# Autodesk Inventor assembly: ensamble_general
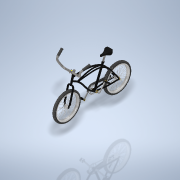
[picture p0: Inventor's stored thumbnail of the model, 180x180]
Saved by Autodesk Inventor 2021 (Build 250183000, 183)
## iProperties
Created: 2021-04-10
Part Number: ensamble_general
Document SubType Name: Assembly
Designer: j2seb
Author: j2seb
## Documents named in this file (17)
- C:\Users\leo7s\Documents\Universidad\03 APM\04 Gitrespository\Proyecto_APM\02 Inventor\ensamble_general.iam
- C:\Users\leo7s\Documents\Universidad\03 APM\04 Gitrespository\Proyecto_APM\02 Inventor\Marco_Bicicleta.iam
- C:\Users\leo7s\Documents\Universidad\03 APM\04 Gitrespository\Proyecto_APM\02 Inventor\Manubrio\Manubrio.ipt
- C:\Users\leo7s\Documents\Universidad\03 APM\04 Gitrespository\Proyecto_APM\02 Inventor\sillin.iam
- C:\Users\leo7s\Documents\Universidad\03 APM\04 Gitrespository\Proyecto_APM\02 Inventor\caja_pedalera.iam
- C:\Users\leo7s\Documents\Universidad\03 APM\04 Gitrespository\Proyecto_APM\02 Inventor\Transmision\Cadena.iam
- C:\Users\leo7s\Documents\Universidad\03 APM\04 Gitrespository\Proyecto_APM\02 Inventor\cubrecadena.ipt
- C:\Users\leo7s\Documents\Universidad\03 APM\04 Gitrespository\Proyecto_APM\02 Inventor\llanta trasera.iam
- C:\Users\leo7s\Documents\Universidad\03 APM\04 Gitrespository\Proyecto_APM\02 Inventor\llanta delantera.iam
- C:\Users\leo7s\Documents\Universidad\03 APM\04 Gitrespository\Proyecto_APM\02 Inventor\platina_1.ipt
- C:\Users\leo7s\Documents\Universidad\03 APM\04 Gitrespository\Proyecto_APM\02 Inventor\platina_2.ipt
- C:\Users\leo7s\Documents\Universidad\03 APM\04 Gitrespository\Proyecto_APM\02 Inventor\platina_3.ipt
- C:\Users\j2seb\OneDrive\Documents\Inventor\Content Center Files\R2021\es-ES\ISO 7045(1)\DIN EN ISO 7045 - M3 x 8 - 4.8 - H.ipt
- C:\Users\j2seb\OneDrive\Documents\Inventor\Content Center Files\R2021\es-ES\DIN 125-2  A\DIN 125-2 - A 3,2A.ipt
- C:\Users\j2seb\OneDrive\Documents\Inventor\Content Center Files\R2021\es-ES\DIN 439-2\DIN 439 - M3 x 0,5.ipt
- C:\Users\j2seb\OneDrive\Documents\Inventor\Content Center Files\R2021\es-ES\ISO 7045(2)\DIN EN ISO 7045 - M3 x 8 - 4.8 - Z.ipt
- C:\Users\leo7s\Documents\Universidad\03 APM\04 Gitrespository\Proyecto_APM\02 Inventor\platina_4.ipt
## Components (21 placed, 16 different names)
1. Marco_Bicicleta:1 [sub-assembly] — Flush:1, Cylindrical:2, Mate:5, Coincidencia:6, Coincidencia:7, Mate:8, Mate:9, Coincidencia:16, Coincidencia:19, Mate:20, Coincidencia:37
2. Manubrio:1 — Flush:1, Coincidencia:19, Mate:21
3. sillin:1 [sub-assembly] — Cylindrical:2, Mate:5
4. caja_pedalera:1 [sub-assembly] — Coincidencia:6, Coincidencia:7
5. Cadena:1 [sub-assembly] — Mate:12
6. cubrecadena:1 — Mate:15, Coincidencia:23, Nivelación:2, Coincidencia:24, Nivelación:3, Coincidencia:25, Coincidencia:29, Coincidencia:30, Coincidencia:31, Coincidencia:32, Nivelación:4
7. llanta trasera:1 [sub-assembly] — Coincidencia:16
8. llanta delantera:1 [sub-assembly] — Mate:20, Mate:22
9. platina_1:1 — Coincidencia:23, Nivelación:2, Coincidencia:26, Coincidencia:27, Coincidencia:28
10. platina_2:1 — Coincidencia:24, Nivelación:3, Nivelación:4, Coincidencia:34
11. platina_3:1 — Coincidencia:25, Coincidencia:33
12. DIN EN ISO 7045 H M3 x 8 - 4.8 - H:1 — Coincidencia:26, Coincidencia:27
13. DIN 125-2 A A 3,2:1 — Coincidencia:28, Coincidencia:29, Insertar:1
14. DIN 439-2 - reemplazado por DIN EN 24035/28675 M3:1 — Insertar:1
15. DIN EN ISO 7045 Z M3 x 8 - 4.8 - Z:1 — Coincidencia:30, Coincidencia:31
16. DIN 125-2 A A 3,2:2 — Coincidencia:32, Coincidencia:33, Insertar:2
17. DIN 439-2 - reemplazado por DIN EN 24035/28675 M3:2 — Insertar:2
18. DIN EN ISO 7045 H M3 x 8 - 4.8 - H:2 — Coincidencia:34, Coincidencia:35, Coincidencia:36
19. DIN 125-2 A A 3,2:3 — Coincidencia:35
20. DIN 439-2 - reemplazado por DIN EN 24035/28675 M3:3 — Coincidencia:36
21. platina_4:1 — Coincidencia:37
## Relationships (35: Mate 28, Flush 4, Insert 2, CylindricalJoint 1)
- [Mate]: Marco_Bicicleta:1 ↔ llanta trasera:1
- Flush:1 (-55.052 mm): Marco_Bicicleta:1 ↔ Manubrio:1
- Cylindrical:2: Marco_Bicicleta:1 ↔ sillin:1
- Mate:5 (-50 mm): Marco_Bicicleta:1 ↔ sillin:1
- Coincidencia:6 [Mate]: Marco_Bicicleta:1 ↔ caja_pedalera:1
- Coincidencia:7 [Mate]: Marco_Bicicleta:1 ↔ caja_pedalera:1
- Mate:8: Marco_Bicicleta:1
- Mate:9: Marco_Bicicleta:1
- Mate:12: Cadena:1
- Mate:15: cubrecadena:1
- Coincidencia:16 [Mate]: Marco_Bicicleta:1 ↔ llanta trasera:1
- Coincidencia:19 [Mate]: Marco_Bicicleta:1 ↔ Manubrio:1
- Mate:20: Marco_Bicicleta:1 ↔ llanta delantera:1
- Mate:21: Manubrio:1
- Mate:22: llanta delantera:1
- Coincidencia:23 [Mate]: cubrecadena:1 ↔ platina_1:1
- Nivelación:2 [Flush]: cubrecadena:1 ↔ platina_1:1
- Coincidencia:24 [Mate]: cubrecadena:1 ↔ platina_2:1
- Nivelación:3 [Flush]: cubrecadena:1 ↔ platina_2:1
- Coincidencia:25 [Mate]: cubrecadena:1 ↔ platina_3:1
- Coincidencia:26 [Mate]: platina_1:1 ↔ DIN EN ISO 7045 H M3 x 8 - 4.8 - H:1
- Coincidencia:27 [Mate]: platina_1:1 ↔ DIN EN ISO 7045 H M3 x 8 - 4.8 - H:1
- Coincidencia:28 [Mate]: platina_1:1 ↔ DIN 125-2 A A 3,2:1
- Coincidencia:29 [Mate]: cubrecadena:1 ↔ DIN 125-2 A A 3,2:1
- Insertar:1: DIN 125-2 A A 3,2:1 ↔ DIN 439-2 - reemplazado por DIN EN 24035/28675 M3:1
- Coincidencia:30 [Mate]: cubrecadena:1 ↔ DIN EN ISO 7045 Z M3 x 8 - 4.8 - Z:1
- Coincidencia:31 [Mate]: cubrecadena:1 ↔ DIN EN ISO 7045 Z M3 x 8 - 4.8 - Z:1
- Coincidencia:32 [Mate]: cubrecadena:1 ↔ DIN 125-2 A A 3,2:2
- Coincidencia:33 [Mate]: platina_3:1 ↔ DIN 125-2 A A 3,2:2
- Insertar:2: DIN 125-2 A A 3,2:2 ↔ DIN 439-2 - reemplazado por DIN EN 24035/28675 M3:2
- Nivelación:4 [Flush]: cubrecadena:1 ↔ platina_2:1
- Coincidencia:34 [Mate]: platina_2:1 ↔ DIN EN ISO 7045 H M3 x 8 - 4.8 - H:2
- Coincidencia:35 [Mate]: DIN EN ISO 7045 H M3 x 8 - 4.8 - H:2 ↔ DIN 125-2 A A 3,2:3
- Coincidencia:36 [Mate]: DIN EN ISO 7045 H M3 x 8 - 4.8 - H:2 ↔ DIN 439-2 - reemplazado por DIN EN 24035/28675 M3:3
- Coincidencia:37 [Mate] (8 mm): Marco_Bicicleta:1 ↔ platina_4:1
## Named parameters: DExtTub = 42.164 mm, DintTub = 35.052 mm, DIntTubTen = 28 mm, DAguUniMarcoLlanta = 5 mm
